# Autodesk Inventor assembly: EnsambleFinal
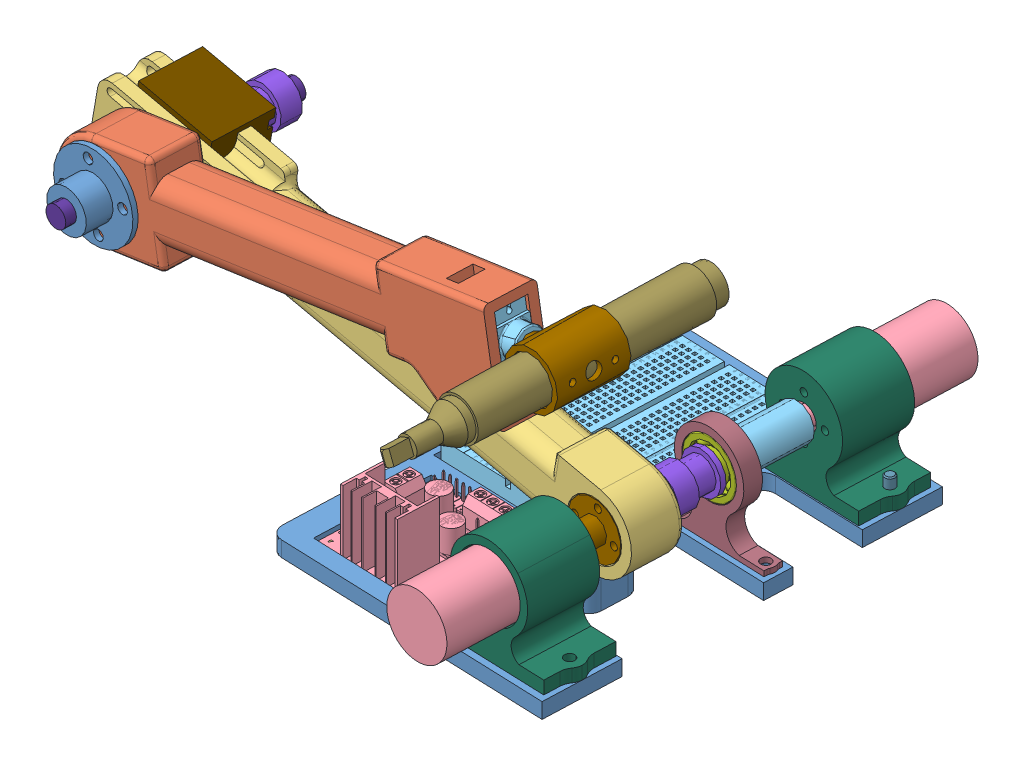
[picture p0: shaded view drawn from the shape stored in the file]
Saved by Autodesk Inventor 2021 (Build 250183000, 183)
## iProperties
Created: 2022-10-27
Part Number: EnsambleFinal
Document SubType Name: Assembly
Designer: zulet
Author: zulet
## Documents named in this file (23)
- D:\UNAL\2022-2S\Servomecanismos\Proyecto Academico\Servomecanismo2R-main\Servomecanismo2R\INVENTOR\Piezas3D\Piezas3D\EnsambleFinal.iam
- D:\UNAL\2022-2S\Servomecanismos\Proyecto Academico\Motorreductor.ipt
- D:\UNAL\2022-2S\Servomecanismos\Proyecto Academico\Acople4a8.ipt
- D:\UNAL\2022-2S\Servomecanismos\Proyecto Academico\Polea.ipt
- D:\UNAL\2022-2S\Servomecanismos\Proyecto Academico\Eje8.ipt
- C:\Users\zulet\OneDrive\Documents\Inventor\Content Center Files\R2021\en-US\BS 290 SKF(20)\BS 290 SKF - SKF 608-2RZ.ipt
- D:\UNAL\2022-2S\Servomecanismos\Proyecto Academico\Servomecanismo2R-main\Servomecanismo2R\INVENTOR\Piezas3D\Piezas3D\Eslabon1.ipt
- D:\UNAL\2022-2S\Servomecanismos\Proyecto Academico\Servomecanismo2R-main\Servomecanismo2R\INVENTOR\Piezas3D\Piezas3D\Eslabon2.ipt
- D:\UNAL\2022-2S\Servomecanismos\Proyecto Academico\Servomecanismo2R-main\Servomecanismo2R\INVENTOR\Piezas3D\Piezas3D\Eje.ipt
- D:\UNAL\2022-2S\Servomecanismos\Proyecto Academico\Servomecanismo2R-main\Servomecanismo2R\INVENTOR\Piezas3D\Piezas3D\Tensor.ipt
- D:\UNAL\2022-2S\Servomecanismos\Proyecto Academico\AcopleBrida4.ipt
- D:\UNAL\2022-2S\Servomecanismos\Proyecto Academico\AcopleBrida8mm.ipt
- D:\UNAL\2022-2S\Servomecanismos\Proyecto Academico\Servomecanismo2R-main\Servomecanismo2R\INVENTOR\Piezas3D\Piezas3D\Tower Pro MG90S Micro servo\Tower Pro MG90S Micro servo.iam
- D:\UNAL\2022-2S\Servomecanismos\Proyecto Academico\Servomecanismo2R-main\Servomecanismo2R\INVENTOR\Piezas3D\Piezas3D\BaseM1.ipt
- D:\UNAL\2022-2S\Servomecanismos\Proyecto Academico\Servomecanismo2R-main\Servomecanismo2R\INVENTOR\Piezas3D\Piezas3D\SoporteMarcador.ipt
- D:\UNAL\2022-2S\Servomecanismos\Proyecto Academico\Servomecanismo2R-main\Servomecanismo2R\INVENTOR\Piezas3D\Piezas3D\PortaMarcador.ipt
- D:\UNAL\2022-2S\Servomecanismos\Proyecto Academico\Servomecanismo2R-main\Servomecanismo2R\INVENTOR\Piezas3D\Piezas3D\SoportePolea.ipt
- D:\UNAL\2022-2S\Servomecanismos\Proyecto Academico\Servomecanismo2R-main\Servomecanismo2R\INVENTOR\Piezas3D\PuenteHL298N.ipt
- D:\UNAL\2022-2S\Servomecanismos\Proyecto Academico\Servomecanismo2R-main\Servomecanismo2R\INVENTOR\Piezas3D\Piezas3D\proto_400.ipt
- D:\UNAL\2022-2S\Servomecanismos\Proyecto Academico\Servomecanismo2R-main\Servomecanismo2R\INVENTOR\Piezas3D\Piezas3D\PlacaBase.ipt
- D:\UNAL\2022-2S\Servomecanismos\Proyecto Academico\Servomecanismo2R-main\Servomecanismo2R\INVENTOR\Piezas3D\Piezas3D\marcador.ipt
- C:\Users\zulet\OneDrive\Documents\Inventor\Content Center Files\R2021\en-US\DIN 6912\DIN 6912 - M4 x 12.ipt
- C:\Users\zulet\OneDrive\Documents\Inventor\Content Center Files\R2021\en-US\DIN 7985 (H)\DIN 7985 (H) - M2x6-H.ipt
## Components (27 placed, 22 different names)
1. Motorreductor:1 — Mate:3, Mate:4, Mate:46, Mate:47
2. Acople4a8:1 — Flush:3, Mate:3, Mate:4, Mate:13, Mate:17, Mate:34
3. Eje8:1 — Flush:3, Mate:13, Mate:14, Mate:16, Mate:33
4. BS 290 SKF- with two low-friction seals SKF 608-2RZ:1 — Mate:5, Mate:6, Mate:16, Flush:6
5. Eslabon1:1 — Mate:5, Mate:6, Mate:7, Mate:8, Flush:5, Mate:18, Flush:7
6. Eslabon2:1 — Mate:12, Mate:18, Flush:8, Flush:9, Flush:10, Mate:21, Mate:22, Mate:23
7. Eje:1 — Mate:10, Mate:11, Mate:12, Flush:11
8. Tensor:1 — Mate:7, Mate:8, Mate:9, Flush:4, Flush:5
9. Polea:2 — Mate:11, Mate:15
10. BS 290 SKF- with two low-friction seals SKF 608-2RZ:2 — Mate:9, Flush:4, Mate:10, Mate:15
11. Polea:3 — Mate:14, Flush:6, Mate:17
12. AcopleBrida4:1 — Flush:7, Mate:19, Mate:20
13. Motorreductor:2 — Mate:19, Mate:20, Mate:48, Mate:49
14. AcopleBrida8mm:1 — Flush:8, Flush:9, Flush:10, Flush:11
15. Tower Pro MG90S Micro servo:1 [sub-assembly] — Mate:21, Mate:22, Mate:23, Flush:13, Mate:24, Mate:57
16. SoporteMarcador:1 — Flush:13
17. PortaMarcador:1 — Mate:24, Mate:29, Flush:20, Mate:56, Mate:57, Mate:58
18. BS 290 SKF- with two low-friction seals SKF 608-2RZ:3 — Mate:30, Flush:21, Mate:33
19. PuenteHL298N:1 — Mate:41, Mate:42, Mate:43
20. proto_400:1 — Mate:38, Mate:39, Mate:40
21. PlacaBase:1 — Mate:38, Mate:39, Mate:40, Mate:41, Mate:42, Mate:43, Mate:44, Mate:50, Mate:51, Mate:53, Mate:54, Mate:55
22. marcador:1 — Mate:29, Flush:20
23. SoportePolea:1 — Mate:30, Flush:21, Mate:34, Mate:53
24. DIN 6912 M4 x 12:1 — Mate:44, Mate:52, Mate:55
25. BaseM1:1 — Mate:46, Mate:47, Mate:50, Mate:51, Mate:52
26. BaseM1:2 — Mate:48, Mate:49, Mate:54
27. DIN 7985 (H) M2x6-H:1 — Mate:56, Mate:58
## Relationships (58: Mate 46, Flush 12)
- Flush:3: Acople4a8:1 ↔ Eje8:1
- Mate:3: Motorreductor:1 ↔ Acople4a8:1
- Mate:4 (2 mm): Motorreductor:1 ↔ Acople4a8:1
- Mate:5: BS 290 SKF- with two low-friction seals SKF 608-2RZ:1 ↔ Eslabon1:1
- Mate:6: BS 290 SKF- with two low-friction seals SKF 608-2RZ:1 ↔ Eslabon1:1
- Mate:7: Eslabon1:1 ↔ Tensor:1
- Mate:8: Eslabon1:1 ↔ Tensor:1
- Mate:9: Tensor:1 ↔ BS 290 SKF- with two low-friction seals SKF 608-2RZ:2
- Flush:4: Tensor:1 ↔ BS 290 SKF- with two low-friction seals SKF 608-2RZ:2
- Flush:5 (-10 mm): Eslabon1:1 ↔ Tensor:1
- Mate:10: Eje:1 ↔ BS 290 SKF- with two low-friction seals SKF 608-2RZ:2
- Mate:11: Eje:1 ↔ Polea:2
- Mate:12: Eslabon2:1 ↔ Eje:1
- Mate:13: Acople4a8:1 ↔ Eje8:1
- Mate:14: Eje8:1 ↔ Polea:3
- Mate:15 (1 mm): Polea:2 ↔ BS 290 SKF- with two low-friction seals SKF 608-2RZ:2
- Mate:16: Eje8:1 ↔ BS 290 SKF- with two low-friction seals SKF 608-2RZ:1
- Flush:6 (12 mm): BS 290 SKF- with two low-friction seals SKF 608-2RZ:1 ↔ Polea:3
- Mate:17 (9 mm): Acople4a8:1 ↔ Polea:3
- Mate:18 (1 mm): Eslabon1:1 ↔ Eslabon2:1
- Flush:7: Eslabon1:1 ↔ AcopleBrida4:1
- Mate:19: AcopleBrida4:1 ↔ Motorreductor:2
- Mate:20 (2 mm): AcopleBrida4:1 ↔ Motorreductor:2
- Flush:8: Eslabon2:1 ↔ AcopleBrida8mm:1
- Flush:9: Eslabon2:1 ↔ AcopleBrida8mm:1
- Flush:10: Eslabon2:1 ↔ AcopleBrida8mm:1
- Flush:11 (-4 mm): Eje:1 ↔ AcopleBrida8mm:1
- Mate:21: Eslabon2:1 ↔ Tower Pro MG90S Micro servo:1
- Mate:22: Eslabon2:1 ↔ Tower Pro MG90S Micro servo:1
- Mate:23: Eslabon2:1 ↔ Tower Pro MG90S Micro servo:1
- Flush:13: Tower Pro MG90S Micro servo:1 ↔ SoporteMarcador:1
- Mate:24: Tower Pro MG90S Micro servo:1 ↔ PortaMarcador:1
- Mate:29: PortaMarcador:1 ↔ marcador:1
- Flush:20 (-40 mm): PortaMarcador:1 ↔ marcador:1
- Mate:30: BS 290 SKF- with two low-friction seals SKF 608-2RZ:3 ↔ SoportePolea:1
- Flush:21: BS 290 SKF- with two low-friction seals SKF 608-2RZ:3 ↔ SoportePolea:1
- Mate:33: Eje8:1 ↔ BS 290 SKF- with two low-friction seals SKF 608-2RZ:3
- Mate:34 (1 mm): Acople4a8:1 ↔ SoportePolea:1
- Mate:38: proto_400:1 ↔ PlacaBase:1
- Mate:39: proto_400:1 ↔ PlacaBase:1
- Mate:40: proto_400:1 ↔ PlacaBase:1
- Mate:41: PuenteHL298N:1 ↔ PlacaBase:1
- Mate:42: PuenteHL298N:1 ↔ PlacaBase:1
- Mate:43: PuenteHL298N:1 ↔ PlacaBase:1
- Mate:44: PlacaBase:1 ↔ DIN 6912 M4 x 12:1
- Mate:46: Motorreductor:1 ↔ BaseM1:1
- Mate:47: Motorreductor:1 ↔ BaseM1:1
- Mate:48: Motorreductor:2 ↔ BaseM1:2
- Mate:49: Motorreductor:2 ↔ BaseM1:2
- Mate:50: PlacaBase:1 ↔ BaseM1:1
- Mate:51: PlacaBase:1 ↔ BaseM1:1
- Mate:52: DIN 6912 M4 x 12:1 ↔ BaseM1:1
- Mate:53: PlacaBase:1 ↔ SoportePolea:1
- Mate:54: PlacaBase:1 ↔ BaseM1:2
- Mate:55: PlacaBase:1 ↔ DIN 6912 M4 x 12:1
- Mate:56: PortaMarcador:1 ↔ DIN 7985 (H) M2x6-H:1
- Mate:57: Tower Pro MG90S Micro servo:1 ↔ PortaMarcador:1
- Mate:58: PortaMarcador:1 ↔ DIN 7985 (H) M2x6-H:1
